# Autodesk Inventor assembly: Ball End
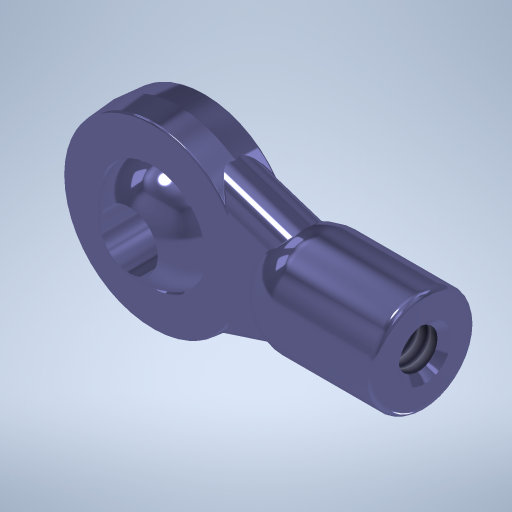
[picture p0: Inventor's stored thumbnail of the model, 512x512]
Saved by Autodesk Inventor 2023.1 (Build 271208000, 208)
## iProperties
Created: 2019-12-01
Part Number: Ball End
Document SubType Name: Assembly
Designer: Jopa
Author: Jopa
## Documents named in this file (3)
- C:\Users\Arzum Naz Doğaner\OneDrive\Masaüstü\HUDSON süspansiyon\Ball End.iam
- C:\Users\Arzum Naz Doğaner\OneDrive\Masaüstü\HUDSON süspansiyon\Ball End.ipt
- C:\Users\Arzum Naz Doğaner\OneDrive\Masaüstü\HUDSON süspansiyon\0.25 Ball.ipt
## Components (2 placed, 2 different names)
1. Ball End:1 — Mate:1, Mate:2
2. 0.25 Ball:1 — Mate:1, Mate:2
## Relationships (2: Mate 2)
- Mate:1: Ball End:1 ↔ 0.25 Ball:1
- Mate:2: Ball End:1 ↔ 0.25 Ball:1
